# Autodesk Inventor assembly: sar340+ couplers
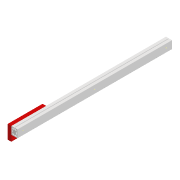
[picture p0: Inventor's stored thumbnail of the model, 180x180]
Saved by Autodesk Inventor 2020 (Build 240168000, 168)
## iProperties
Created: 2019-11-23
Part Number: sar340+ couplers
Document SubType Name: Assembly
Designer: ball
Author: ball
## Documents named in this file (3)
- C:\FTC\FTC8863CAD\2019 Robot\Delivery\extension arm\sar340+ couplers.iam
- C:\FTC\FTC8863CAD\Misumi\SAR340\SAR340.iam
- C:\FTC\FTC8863CAD\2019 Robot\Delivery\Coupler collector regular.ipt
## Components (2 placed, 2 different names)
1. SAR340:1 [sub-assembly] — Mate:1, Mate:2, Flush:1
2. Coupler collector regular:1 — Mate:1, Mate:2, Flush:1
## Relationships (3: Mate 2, Flush 1)
- Mate:1: SAR340:1 ↔ Coupler collector regular:1
- Mate:2: SAR340:1 ↔ Coupler collector regular:1
- Flush:1: SAR340:1 ↔ Coupler collector regular:1
